# Autodesk Inventor assembly: Encoder-Motor-Llanta
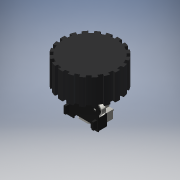
[picture p0: Inventor's stored thumbnail of the model, 180x180]
Saved by Autodesk Inventor 2017 (Build 210142000, 142)
## iProperties
Part Number: Encoder-Motor-Llanta
Material: Genérico
Document SubType Name: Assembly
Designer: fam
Author: fam
## Documents named in this file (4)
- C:\Users\fam\Desktop\UVG\Ciclo 9\Megaproyecto\Megaproyecto\Diseños Inventor Fase 2\Encoder-Motor-Llanta.iam
- C:\Users\fam\Desktop\UVG\Ciclo 9\Megaproyecto\Megaproyecto\Diseños Inventor Fase 2\Encoder.ipt
- C:\Users\fam\Desktop\UVG\Ciclo 9\Megaproyecto\Megaproyecto\Diseños Inventor Fase 2\Motor.ipt
- C:\Users\fam\Desktop\UVG\Ciclo 9\Megaproyecto\Megaproyecto\Diseños Inventor Fase 2\Llanta.ipt
## Components (3 placed, 3 different names)
1. Encoder:1 — Coincidencia:1, Coincidencia:2, Coincidencia:3
2. Motor:1 — Coincidencia:1, Coincidencia:2, Coincidencia:3, Coincidencia:4, Coincidencia:5
3. Llanta:1 — Coincidencia:4, Coincidencia:5
## Relationships (5: Mate 5)
- Coincidencia:1 [Mate]: Encoder:1 ↔ Motor:1
- Coincidencia:2 [Mate]: Encoder:1 ↔ Motor:1
- Coincidencia:3 [Mate]: Encoder:1 ↔ Motor:1
- Coincidencia:4 [Mate]: Motor:1 ↔ Llanta:1
- Coincidencia:5 [Mate] (-45.5 mm): Motor:1 ↔ Llanta:1
